# Autodesk Inventor assembly: MotorAssembly
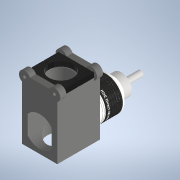
[picture p0: Inventor's stored thumbnail of the model, 180x180]
Saved by Autodesk Inventor 2022 (Build 260153000, 153)
## iProperties
Created: 2022-02-05
Part Number: MotorAssembly
Document SubType Name: Assembly
Designer: ultra
Author: ultra
## Documents named in this file (5)
- C:\Users\ultra\Desktop\Github\RASA-Drone\CAD Files\Drone\MotorAssembly.iam
- C:\Users\ultra\Desktop\Github\RASA-Drone\CAD Files\Drone\KDE2814XF-SERIES.iam
- C:\Users\ultra\Desktop\Github\RASA-Drone\CAD Files\Drone\MotorAdaptor.ipt
- C:\Users\ultra\Desktop\Github\RASA-Drone\CAD Files\Drone\MotorMount.ipt
- C:\Users\ultra\Desktop\Github\RASA-Drone\CAD Files\Drone\TubeClamp.ipt
## Components (5 placed, 4 different names)
1. KDE2814XF-SERIES:1 [sub-assembly] — Insert:1, Insert:2
2. MotorAdaptor:1 — Insert:1
3. MotorMount:1 — Insert:2, Angle:1, Insert:3, Insert:4, Angle:2, Angle:3
4. TubeClamp:1 — Angle:1, Insert:3, Flush:1
5. TubeClamp:2 — Insert:4, Flush:1, Angle:2
## Relationships (8: Insert 4, Angle 3, Flush 1)
- Insert:1: KDE2814XF-SERIES:1 ↔ MotorAdaptor:1
- Insert:2: KDE2814XF-SERIES:1 ↔ MotorMount:1
- Angle:1 (0 deg): MotorMount:1 ↔ TubeClamp:1
- Insert:3: MotorMount:1 ↔ TubeClamp:1
- Insert:4: MotorMount:1 ↔ TubeClamp:2
- Flush:1: TubeClamp:1 ↔ TubeClamp:2
- Angle:2 (0 deg): MotorMount:1 ↔ TubeClamp:2
- Angle:3 (0 deg): MotorMount:1
